# Autodesk Inventor assembly: Assembly
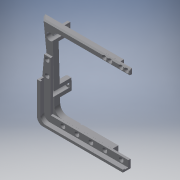
[picture p0: Inventor's stored thumbnail of the model, 180x180]
Saved by Autodesk Inventor 2017 (Build 210142000, 142)
## iProperties
Created: 2022-11-18
Part Number: Assembly
Document SubType Name: Assembly
Designer: khonsu
Author: khonsu
## Documents named in this file (5)
- C:\Users\khonsu\Desktop\Assembly.iam
- C:\Users\khonsu\Desktop\iPadGolf6Holder.ipt
- C:\Users\khonsu\Desktop\iPadGolf6HolderMount.ipt
- C:\Users\khonsu\Desktop\topSpacer.ipt
- C:\Users\khonsu\Desktop\bottomSpacer.ipt
## Components (4 placed, 4 different names)
1. iPadGolf6Holder:1 — Mate:1, Mate:2, Mate:3, Flush:1, Flush:2, Mate:4, Mate:5
2. iPadGolf6HolderMount:1 — Mate:1, Mate:2, Mate:3, Flush:3, Mate:6
3. topSpacer:1 — Flush:1, Flush:2, Mate:4
4. bottomSpacer:1 — Mate:5, Flush:3, Mate:6
## Relationships (9: Mate 6, Flush 3)
- Mate:1: iPadGolf6Holder:1 ↔ iPadGolf6HolderMount:1
- Mate:2: iPadGolf6Holder:1 ↔ iPadGolf6HolderMount:1
- Mate:3: iPadGolf6Holder:1 ↔ iPadGolf6HolderMount:1
- Flush:1: iPadGolf6Holder:1 ↔ topSpacer:1
- Flush:2: iPadGolf6Holder:1 ↔ topSpacer:1
- Mate:4: iPadGolf6Holder:1 ↔ topSpacer:1
- Mate:5: iPadGolf6Holder:1 ↔ bottomSpacer:1
- Flush:3: iPadGolf6HolderMount:1 ↔ bottomSpacer:1
- Mate:6: iPadGolf6HolderMount:1 ↔ bottomSpacer:1
